# Autodesk Inventor assembly: mini predator camera block for boolian
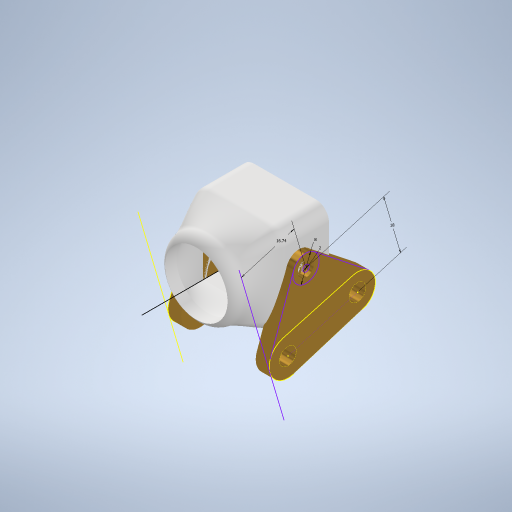
[picture p0: Inventor's stored thumbnail of the model, 512x512]
Saved by Autodesk Inventor 2023 (Build 270158000, 158)
## iProperties
Created: 2023-02-19
Part Number: mini predator camera block for boolian
Document SubType Name: Assembly
Designer: Steven
Author: Steven
## Documents named in this file (5)
- Y:\FPV drone stuff\0 Street League\Frames\PB-Kauri-X\3D prints\35 mm canopy\work in progress prints\Camera mounts\predator mini\mini predator camera block for boolian.iam
- Y:\FPV drone stuff\0 Street League\Frames\PB-Kauri-X\3D prints\35 mm canopy\work in progress prints\Camera mounts\predator mini\mini predator camera block.ipt
- Y:\FPV drone stuff\0 Street League\Frames\PB-Kauri-X\3D prints\35 mm canopy\work in progress prints\Camera mounts\predator mini\mini predator dummy camera.ipt
- Y:\FPV drone stuff\0 Street League\Frames\PB-Kauri-X\3D prints\35 mm canopy\work in progress prints\Camera mounts\Kauri modular camera mount mini.ipt
- Y:\FPV drone stuff\0 Street League\Frames\PB-Kauri-X\3D prints\35 mm canopy\work in progress prints\Camera mounts\predator mini\adjustable camera mount mirror.ipt
## Components (4 placed, 4 different names)
1. mini predator camera block:1 — Flush:1, Flush:2, Flush:3, Flush:4, Flush:5, Flush:6, Mate:1, Mate:2, Flush:7, Angle:1
2. mini predator dummy camera:1 — Flush:4, Flush:5, Flush:6
3. Kauri modular camera mount mini:1 — Mate:1, Mate:2, Mate:3, Mate:4
4. adjustable camera mount mirror:1 — Mate:3, Mate:4, Flush:7, Angle:1
## Relationships (12: Flush 7, Mate 4, Angle 1)
- Flush:1: mini predator camera block:1
- Flush:2: mini predator camera block:1
- Flush:3: mini predator camera block:1
- Flush:4 (2 mm): mini predator camera block:1 ↔ mini predator dummy camera:1
- Flush:5 (2 mm): mini predator camera block:1 ↔ mini predator dummy camera:1
- Flush:6: mini predator camera block:1 ↔ mini predator dummy camera:1
- Mate:1 (-2 mm): mini predator camera block:1 ↔ Kauri modular camera mount mini:1
- Mate:2: mini predator camera block:1 ↔ Kauri modular camera mount mini:1
- Mate:3: Kauri modular camera mount mini:1 ↔ adjustable camera mount mirror:1
- Mate:4: Kauri modular camera mount mini:1 ↔ adjustable camera mount mirror:1
- Flush:7: mini predator camera block:1 ↔ adjustable camera mount mirror:1
- Angle:1 (196.45 deg): mini predator camera block:1 ↔ adjustable camera mount mirror:1
